# Autodesk Inventor assembly: mascon-new
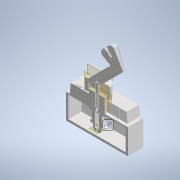
[picture p0: Inventor's stored thumbnail of the model, 180x180]
Saved by Autodesk Inventor 2022 (Build 260153000, 153)
## iProperties
Created: 2021-04-28
Part Number: mascon-new
Document SubType Name: Assembly
Designer: ben
Author: ben
## Documents named in this file (9)
- C:\Users\teh18\Documents\GitHub\r68-bve-mascon\mascon-new.iam
- C:\Users\teh18\Documents\GitHub\r68-bve-mascon\handle\handle.iam
- C:\Users\teh18\Documents\GitHub\r68-bve-mascon\shell\shell.iam
- C:\Users\teh18\Documents\GitHub\r68-bve-mascon\handle_holder.ipt
- C:\Users\teh18\Documents\GitHub\r68-bve-mascon\Reverser.ipt
- C:\Users\teh18\Documents\GitHub\r68-bve-mascon\handle-base\handle_base.iam
- C:\Users\teh18\Documents\GitHub\r68-bve-mascon\handle_base2.ipt
- C:\Users\teh18\Documents\GitHub\r68-bve-mascon\handle-base\PotAttachment.ipt
- C:\Users\teh18\Documents\GitHub\r68-bve-mascon\handle-base\SpringRod.ipt
## Components (8 placed, 8 different names)
1. shell:1 [sub-assembly] — Flush:4, Mate:29, Mate:30
2. handle_holder:1
3. Reverser:1 — Flush:4
4. handle:1 [sub-assembly]
5. handle_base:1 [sub-assembly] — Mate:29, Mate:30, Mate:34, Mate:35, Mate:36
6. handle_base2:1 — Mate:28, Mate:34, Mate:35, Mate:36
7. PotAttachment:1 — Mate:28
8. SpringRod:1
## Relationships (7: Mate 6, Flush 1)
- Flush:4: shell:1 ↔ Reverser:1
- Mate:28: handle_base2:1 ↔ PotAttachment:1
- Mate:29: shell:1 ↔ handle_base:1
- Mate:30: shell:1 ↔ handle_base:1
- Mate:34: handle_base:1 ↔ handle_base2:1
- Mate:35: handle_base:1 ↔ handle_base2:1
- Mate:36: handle_base:1 ↔ handle_base2:1
